# Autodesk Inventor assembly: quick-start-plus4
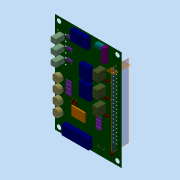
[picture p0: Inventor's stored thumbnail of the model, 180x180]
Saved by Autodesk Inventor 2013 (Build 170138000, 138)
## iProperties
Created: 2013-01-27
Part Number: quick-start-plus4
Document SubType Name: Assembly
Designer: davidgitz
Author: davidgitz
## Documents named in this file (11)
- C:\SharedDrive\Dropbox\ICARUS\Flyer\v4\Mechanical\v4RevA.2\FuselageAssy\Secondary Controller\FAST Robotics, Daughterboard\quick-start-plus4.iam
- C:\SharedDrive\Dropbox\ICARUS\Flyer\v4\Mechanical\v4RevA.2\FuselageAssy\Secondary Controller\FAST Robotics, Daughterboard\quick-start-plus_Outline4.ipt
- C:\SharedDrive\Dropbox\ICARUS\Flyer\v4\Mechanical\v4RevA.2\FuselageAssy\Secondary Controller\FAST Robotics, Daughterboard\SOIC16-N_MC, MCP3208-XX_SL_14.ipt
- C:\SharedDrive\Dropbox\ICARUS\Flyer\v4\Mechanical\v4RevA.2\FuselageAssy\Secondary Controller\FAST Robotics, Daughterboard\3, 3WP_34.ipt
- C:\SharedDrive\Dropbox\ICARUS\Flyer\v4\Mechanical\v4RevA.2\FuselageAssy\Secondary Controller\FAST Robotics, Daughterboard\2, 2WP_124.ipt
- C:\SharedDrive\Dropbox\ICARUS\Flyer\v4\Mechanical\v4RevA.2\FuselageAssy\Secondary Controller\FAST Robotics, Daughterboard\0805, RA-SM_244.ipt
- C:\SharedDrive\Dropbox\ICARUS\Flyer\v4\Mechanical\v4RevA.2\FuselageAssy\Secondary Controller\FAST Robotics, Daughterboard\LEDT175, LED_284.ipt
- C:\SharedDrive\Dropbox\ICARUS\Flyer\v4\Mechanical\v4RevA.2\FuselageAssy\Secondary Controller\FAST Robotics, Daughterboard\4, 4WP_334.ipt
- C:\SharedDrive\Dropbox\ICARUS\Flyer\v4\Mechanical\v4RevA.2\FuselageAssy\Secondary Controller\FAST Robotics, Daughterboard\R-PDSO-G20, TXB0108PWR_354.ipt
- C:\SharedDrive\Dropbox\ICARUS\Flyer\v4\Mechanical\v4RevA.2\FuselageAssy\Secondary Controller\FAST Robotics, Daughterboard\SM0603, 0603YC104KATDA_484.ipt
- C:\SharedDrive\Dropbox\ICARUS\Flyer\v4\Mechanical\v4RevA.2\FuselageAssy\Secondary Controller\FAST Robotics, Daughterboard\FSM2JH, Pushbutton_604.ipt
## Components (55 placed, 55 different names)
1. quick-start-plus_Outline:1 — Mate:4
2. U1_2
3. ANA1_4
4. ANA2_5
5. ANA3_6
6. ANA4_7
7. ANA5_8
8. ANA6_9
9. ANA7_10
10. ANA8_11
11. EPWR1_13
12. SRV1_16
13. SRV2_17
14. SRV3_18
15. SRV4_19
16. US1_20
17. US2_21
18. US3_22
19. US4_23
20. R1_25
21. R2_26
22. R5_27
23. LED1_29
24. LED2_30
25. LED3_31
26. LED4_32
27. UART1_34
28. U2_36
29. U3_37
30. GPIO1_38
31. GPIO2_39
32. GPIO3_40
33. GPIO4_41
34. GPIO5_42
35. U4_43
36. R6_44
37. R7_45
38. R8_46
39. R9_47
40. C1_49
41. C2_50
42. C3_51
43. C4_52
44. C5_55
45. C6_56
46. C7_57
47. C8_58
48. C9_59
49. SW1_61
50. SW2_62
51. SW5_63
52. R3_64
53. R4_65
54. R10_66
55. R11_67
## Relationships (3: Mate 3)
- Mate:2
- Mate:3
- Mate:4: quick-start-plus_Outline:1
